# Autodesk Inventor assembly: Soyuz Stage 2 Core Booster
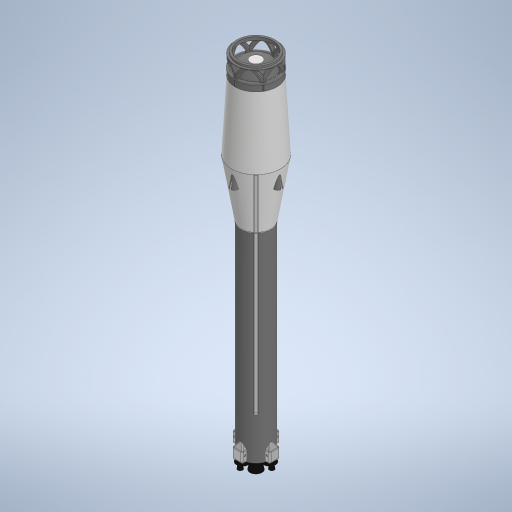
[picture p0: Inventor's stored thumbnail of the model, 512x512]
Saved by Autodesk Inventor 2023 (Build 270158030, 158C)
## iProperties
Created: 2023-01-06
Part Number: Soyuz Stage 2 Core Booster
Document SubType Name: Assembly
Designer: Imogen Heard
Author: Imogen Heard
## Documents named in this file (4)
- C:\Users\dheard\Documents\Inventor\Inventor_Projects\Soyuz Model\Soyuz Stage 2 Core Booster.iam
- C:\Users\dheard\Documents\Inventor\Inventor_Projects\Soyuz Model\Stage2 Core Booster.ipt
- C:\Users\dheard\Documents\Inventor\Inventor_Projects\Soyuz Model\Core Booster Part B.ipt
- C:\Users\dheard\Documents\Inventor\Inventor_Projects\Soyuz Model\Interstage1.ipt
## Components (3 placed, 3 different names)
1. Stage2 Core Booster:1 — Insert:1
2. Core Booster Part B:1 — Insert:1, Insert:2
3. Interstage1:1 — Insert:2
## Relationships (2: Insert 2)
- Insert:1: Stage2 Core Booster:1 ↔ Core Booster Part B:1
- Insert:2: Core Booster Part B:1 ↔ Interstage1:1
